# Autodesk Inventor assembly: Full Wheel Assembly
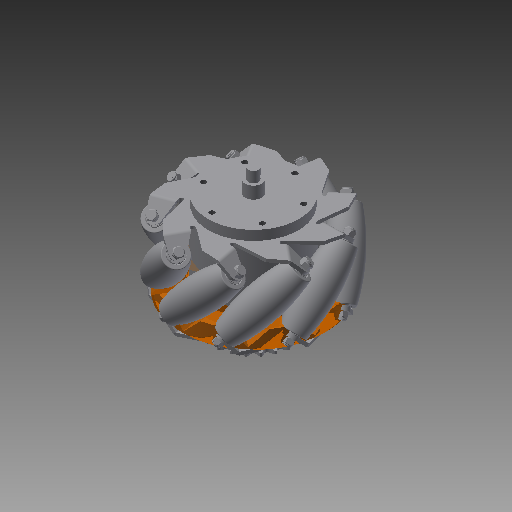
[picture p0: Inventor's stored thumbnail of the model, 512x512]
Saved by Autodesk Inventor 2017 (Build 210142000, 142)
## iProperties
Created: 2017-07-29
Part Number: Full Wheel Assembly
Document SubType Name: Assembly
Designer: User
Author: User
## Documents named in this file (6)
- C:\Robotics\CAD\2016-17_CAD\DriveTrain\wheel sub assembly mechanum wheels .iam
- C:\Robotics\CAD\2016-17_CAD\Mecanum Wheel Adapter.ipt
- C:\Robotics\CAD\COTSParts\Wheels\AndyMark Mecanum Wheels\100mm Aluminum Mecanum wheels.ipt
- C:\Robotics\CAD\2016-17_CAD\Mecanum Wheel Adapter Plate.ipt
- C:\Robotics\CAD\COTSParts\Actobotics\634 parts\634080.ipt
- C:\Robotics\CAD\COTSParts\Actobotics\615 parts\615106.ipt
## Components (5 placed, 5 different names)
1. Mecanum Wheel Adapter:1 — Insert:5, Mate:1, Mate:5
2. 100mm Aluminum Mecanum wheels:1 — Mate:1, Mate:2
3. Mecanum Wheel Adapter Plate:1 — Insert:5, Mate:2, Mate:3
4. 634080:1 — Mate:3, Mate:4
5. 615106:1 — Mate:4, Mate:5
## Relationships (6: Mate 5, Insert 1)
- Insert:5: Mecanum Wheel Adapter:1 ↔ Mecanum Wheel Adapter Plate:1
- Mate:1: Mecanum Wheel Adapter:1 ↔ 100mm Aluminum Mecanum wheels:1
- Mate:2: 100mm Aluminum Mecanum wheels:1 ↔ Mecanum Wheel Adapter Plate:1
- Mate:3: Mecanum Wheel Adapter Plate:1 ↔ 634080:1
- Mate:4: 634080:1 ↔ 615106:1
- Mate:5 (6.35 mm): Mecanum Wheel Adapter:1 ↔ 615106:1
